# Autodesk Inventor assembly: AS_Мехатрон R1
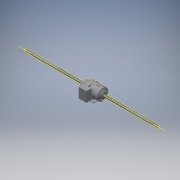
[picture p0: Inventor's stored thumbnail of the model, 180x180]
Saved by Autodesk Inventor 2016 SP1 (Build 200210100, 210)
## iProperties
Created: 2016-04-25
Part Number: AS_Мехатрон R1
Material: Типовые
Document SubType Name: Assembly
Designer: AS
Author: AS
## Documents named in this file (15)
- H:\Projects\GitHub\mechatron\AS_Мехатрон R1.iam
- H:\Projects\GitHub\mechatron\Vint.ipt
- H:\Projects\GitHub\mechatron\2 крышка.ipt
- H:\Projects\GitHub\mechatron\Деталь 3.ipt
- H:\Projects\GitHub\mechatron\Деталь 4.ipt
- H:\Projects\GitHub\mechatron\Деталь 5.ipt
- H:\Projects\GitHub\mechatron\Деталь 6.ipt
- H:\Projects\GitHub\mechatron\Полый вал.iam
- H:\Projects\GitHub\mechatron\Корпус 1 сборка.iam
- H:\Projects\GitHub\mechatron\AS_Мехатрон R1\Мастер проектирования\Болтовое соединение1.iam
- H:\Projects\GitHub\mechatron\AS_Мехатрон R1\Мастер проектирования\Болтовое соединение3.iam
- H:\Projects\GitHub\mechatron\AS_Мехатрон R1\Мастер проектирования\Болтовое соединение4.iam
- H:\Projects\GitHub\mechatron\AS_Мехатрон R1\Мастер проектирования\Болтовое соединение5.iam
- H:\Projects\GitHub\mechatron\fileset\Libraries\Content Center Files\ru-RU\Bearing GOST 27365-87\Подшипник 2007116A ГОСТ 27365-87.ipt
- H:\Projects\GitHub\mechatron\fileset\Libraries\Content Center Files\ru-RU\Bearing GOST 27365-87\Подшипник 2007113A ГОСТ 27365-87.ipt
## Components (32 placed, 11 different names)
1. Vint:1 — Совмещение:1
2. 2 крышка:1 — Заподлицо:2, Совмещение:3, Совмещение:11, Совмещение:15, Совмещение:27, Совмещение:28, Совмещение:30
3. Деталь 3:1 — Совмещение:4, Совмещение:16, Совмещение:17, Заподлицо:11, Совмещение:21, Совмещение:22, Совмещение:32
4. Деталь 4:1 — Заподлицо:5, Совмещение:5, Совмещение:7, Совмещение:17, Совмещение:18
5. Деталь 5:1 — Совмещение:6, Совмещение:11, Совмещение:12, Заподлицо:10, Совмещение:25, Совмещение:26
6. Деталь 6:1 — Заподлицо:7, Совмещение:7, Совмещение:18, Совмещение:23, Совмещение:24
7. Полый вал:1 [sub-assembly] — Совмещение:9, Совмещение:12, Заподлицо:10, Совмещение:29, Совмещение:33, Совмещение:34
8. Корпус 1 сборка:1 [sub-assembly] — Совмещение:10, Заподлицо:8, Заподлицо:9, Совмещение:15, Совмещение:16, Заподлицо:11
9. Подшипник ГОСТ 27365-87 2007116A:1 — Совмещение:29, Совмещение:30
10. Подшипник ГОСТ 27365-87 2007113A:1 — Совмещение:32, Совмещение:33, Совмещение:34
11. Болтовое соединение:1 [sub-assembly] — Совмещение:25, Совмещение:26
12. Болтовое соединение:2 [sub-assembly]
13. Болтовое соединение:3 [sub-assembly]
14. Болтовое соединение:4 [sub-assembly]
15. Болтовое соединение:5 [sub-assembly] — Совмещение:27, Совмещение:28
16. Болтовое соединение:6 [sub-assembly]
17. Болтовое соединение:7 [sub-assembly]
18. Болтовое соединение:8 [sub-assembly]
19. Болтовое соединение:9 [sub-assembly]
20. Болтовое соединение:10 [sub-assembly]
21. Болтовое соединение:11 [sub-assembly] — Совмещение:21, Совмещение:22
22. Болтовое соединение:12 [sub-assembly]
23. Болтовое соединение:13 [sub-assembly]
24. Болтовое соединение:14 [sub-assembly]
25. Болтовое соединение:15 [sub-assembly]
26. Болтовое соединение:16 [sub-assembly]
27. Болтовое соединение:17 [sub-assembly] — Совмещение:23, Совмещение:24
28. Болтовое соединение:18 [sub-assembly]
29. Болтовое соединение:19 [sub-assembly]
30. Болтовое соединение:20 [sub-assembly]
31. Болтовое соединение:21 [sub-assembly]
32. Болтовое соединение:22 [sub-assembly]
## Component patterns: (4 elements, first: Болтовое соединение:1), (6 elements, first: Болтовое соединение:5), (6 elements, first: Болтовое соединение:11), (6 elements, first: Болтовое соединение:17)
## Relationships (34: Mate 27, Flush 7)
- Совмещение:1 [Mate]: Vint:1
- Заподлицо:2 [Flush]: 2 крышка:1
- Совмещение:3 [Mate]: 2 крышка:1
- Совмещение:4 [Mate]: Деталь 3:1
- Заподлицо:5 [Flush]: Деталь 4:1
- Совмещение:5 [Mate]: Деталь 4:1
- Совмещение:6 [Mate]: Деталь 5:1
- Заподлицо:7 [Flush]: Деталь 6:1
- Совмещение:7 [Mate]: Деталь 4:1 ↔ Деталь 6:1
- Совмещение:9 [Mate]: Полый вал:1
- Совмещение:10 [Mate]: Корпус 1 сборка:1
- Заподлицо:8 [Flush]: Корпус 1 сборка:1
- Заподлицо:9 [Flush]: Корпус 1 сборка:1
- Совмещение:11 [Mate]: 2 крышка:1 ↔ Деталь 5:1
- Совмещение:12 [Mate]: Деталь 5:1 ↔ Полый вал:1
- Заподлицо:10 [Flush]: Деталь 5:1 ↔ Полый вал:1
- Совмещение:15 [Mate]: 2 крышка:1 ↔ Корпус 1 сборка:1
- Совмещение:16 [Mate]: Деталь 3:1 ↔ Корпус 1 сборка:1
- Совмещение:17 [Mate]: Деталь 3:1 ↔ Деталь 4:1
- Совмещение:18 [Mate]: Деталь 4:1 ↔ Деталь 6:1
- Заподлицо:11 [Flush]: Деталь 3:1 ↔ Корпус 1 сборка:1
- Совмещение:21 [Mate]: Деталь 3:1 ↔ Болтовое соединение:11
- Совмещение:22 [Mate]: Деталь 3:1 ↔ Болтовое соединение:11
- Совмещение:23 [Mate]: Деталь 6:1 ↔ Болтовое соединение:17
- Совмещение:24 [Mate]: Деталь 6:1 ↔ Болтовое соединение:17
- Совмещение:25 [Mate]: Деталь 5:1 ↔ Болтовое соединение:1
- Совмещение:26 [Mate]: Деталь 5:1 ↔ Болтовое соединение:1
- Совмещение:27 [Mate]: 2 крышка:1 ↔ Болтовое соединение:5
- Совмещение:28 [Mate]: 2 крышка:1 ↔ Болтовое соединение:5
- Совмещение:29 [Mate]: Полый вал:1 ↔ Подшипник ГОСТ 27365-87 2007116A:1
- Совмещение:30 [Mate]: 2 крышка:1 ↔ Подшипник ГОСТ 27365-87 2007116A:1
- Совмещение:32 [Mate]: Деталь 3:1 ↔ Подшипник ГОСТ 27365-87 2007113A:1
- Совмещение:33 [Mate]: Полый вал:1 ↔ Подшипник ГОСТ 27365-87 2007113A:1
- Совмещение:34 [Mate]: Полый вал:1 ↔ Подшипник ГОСТ 27365-87 2007113A:1
